# Autodesk Inventor assembly: PCB_ASSY
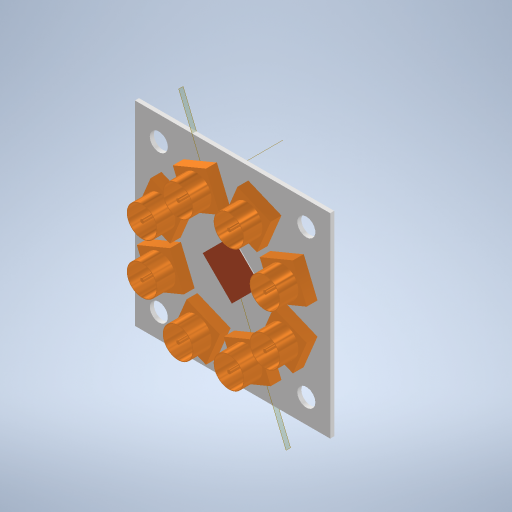
[picture p0: Inventor's stored thumbnail of the model, 512x512]
Saved by Autodesk Inventor 2023.1 (Build 271208000, 208)
## iProperties
Company: Aalto University / OtaNano
Created: 2023-05-15
Part Number: PCB_ASSY
Document SubType Name: Assembly
Designer: Joel Salminen
Author: Joel Salminen
## Documents named in this file (4)
- C:\Users\salminj3\OneDrive - Aalto University\_3D\NANO\Ekaterina Mukhanova\PCB holder\Sent to client on 230817\PCB_ASSY.iam
- C:\Users\salminj3\OneDrive - Aalto University\_3D\NANO\Ekaterina Mukhanova\PCB holder\PCB.ipt
- C:\Users\salminj3\OneDrive - Aalto University\_3D\NANO\Ekaterina Mukhanova\PCB holder\Connector.ipt
- C:\Users\salminj3\OneDrive - Aalto University\_3D\NANO\Ekaterina Mukhanova\PCB holder\Connector_MIR.ipt
## Components (9 placed, 3 different names)
1. PCB:1 — Mate:1, Mate:2, Angle:1
2. Connector:1 — Mate:1, Mate:2, Angle:1
3. Connector_MIR:1
4. Connector:2
5. Connector_MIR:2
6. Connector:3
7. Connector_MIR:3
8. Connector:4
9. Connector_MIR:4
## Component patterns: (4 elements, first: Connector:1 + Connector_MIR:1)
## Relationships (3: Mate 2, Angle 1)
- Mate:1: PCB:1 ↔ Connector:1
- Mate:2: PCB:1 ↔ Connector:1
- Angle:1 (0 deg): PCB:1 ↔ Connector:1
